# Autodesk Inventor assembly: Outer
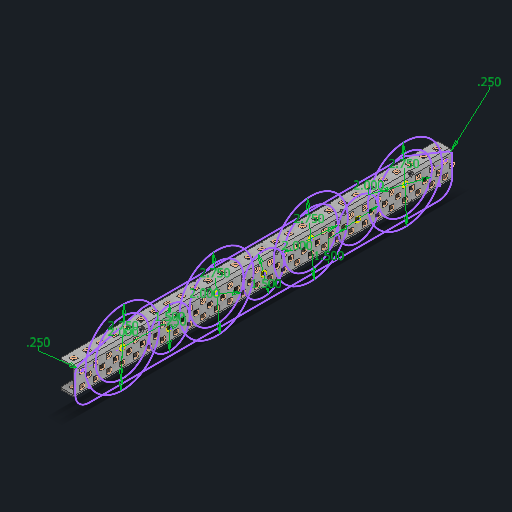
[picture p0: Inventor's stored thumbnail of the model, 512x512]
Saved by Autodesk Inventor 2025.1 (Build 291241000, 241)
## iProperties
Created: 2024-12-17
Part Number: Outer
Document SubType Name: Assembly
Designer: avere
Author: avere
## Documents named in this file (2)
- C:\Users\avere\VEX\High Stakes\CAD\V4\Chassis\Drivebay Left\Outer.iam
- C:\Users\avere\VEX\High Stakes\CAD\ROBOPROS-CAD-Inventor\Structure\C Channel\Aluminum 1x2x1\Alu C 1x2x1x28.ipt
## Components (1 placed, 1 different names)
1. Alu C 1x2x1x28:1 — Flush:1, Flush:2, Flush:3
## Relationships (3: Flush 3)
- Flush:1 (-177.8 mm): Alu C 1x2x1x28:1
- Flush:2 (-12.7 mm): Alu C 1x2x1x28:1
- Flush:3 (-7.9375 mm): Alu C 1x2x1x28:1
